# Autodesk Inventor assembly: DD
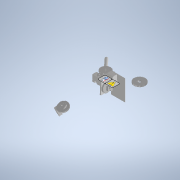
[picture p0: Inventor's stored thumbnail of the model, 180x180]
Saved by Autodesk Inventor 2020.2 (Build 242310000, 310)
## iProperties
Created: 2022-10-31
Part Number: DD
Document SubType Name: Assembly
Designer: Administrator
Author: Administrator
## Documents named in this file (14)
- C:\Users\Administrator\Documents\kamuy2\DD.iam
- C:\Users\Administrator\Documents\kamuy2\Parts\Part1.ipt
- C:\Users\Administrator\Documents\kamuy2\Parts\x-540_idle.ipt
- C:\Users\Administrator\Documents\kamuy2\Parts\XW540.N105.I101.ipt
- C:\Users\Administrator\Documents\kamuy2\Parts\GEABP1.0-80-10-A-20-KFC30-K3_Autodesk_Inventor_2020_20221101\AIS2020\GEABP1_0-80-10-A-20-KFC30-K3.iam
- C:\Users\Administrator\Documents\kamuy2\Parts\GEABP1.0-32-10-A-12-KFC22-K3_Autodesk_Inventor_2020_20221101\AIS2020\GEABP1_0-32-10-A-12-KFC22-K3.iam
- C:\Users\Administrator\Documents\kamuy2\Parts\Part2.ipt
- C:\Users\Administrator\Documents\kamuy2\Parts\Part5.ipt
- C:\Users\Administrator\Documents\kamuy2\Parts\BGHK6800VV-20_Autodesk_Inventor_2020_20221102\AIS2020\BGHK6800VV-20.iam
- C:\Users\Administrator\Documents\kamuy2\Parts\GEABP1.0-70-10-B-10-KFC30-K3_Autodesk_Inventor_2020_20221102\AIS2020\GEABP1_0-70-10-B-10-KFC30-K3.iam
- C:\Users\Administrator\Documents\kamuy2\Parts\Part7.ipt
- C:\Users\Administrator\Documents\kamuy2\Parts\C-SHA10_Autodesk_Inventor_2020_20221104\AIS2020\C-SHA10.iam
- C:\Users\Administrator\Documents\kamuy2\Parts\BGBFS6900DD-25_Autodesk_Inventor_2020_20221104\AIS2020\BGBFS6900DD-25.iam
- C:\Users\Administrator\Documents\kamuy2\Parts\Part8.ipt
## Components (20 placed, 13 different names)
1. Part1:1 — フラッシュ:1, メイト:1, フラッシュ:14, メイト:13, フラッシュ:15
2. x-540_idle:1 — メイト:4, メイト:5, メイト:33, フラッシュ:25, フラッシュ:26, メイト:47, フラッシュ:32
3. XW540.N105.I101:1 — フラッシュ:1, メイト:1, メイト:2, メイト:3, フラッシュ:14, メイト:19
4. GEABP1_0-32-10-A-12-KFC22-K3:1 [sub-assembly] — メイト:2, メイト:3, フラッシュ:22
5. GEABP1_0-32-10-A-12-KFC22-K3:2 [sub-assembly] — メイト:4, メイト:5, フラッシュ:23
6. Part2:1
7. x-540_idle:2
8. GEABP1_0-32-10-A-12-KFC22-K3:3 [sub-assembly] — フラッシュ:24
9. GEABP1_0-80-10-A-20-KFC30-K3:4 [sub-assembly]
10. Part5:1 — メイト:25, メイト:26, メイト:27, メイト:33, フラッシュ:25, フラッシュ:26, メイト:43, フラッシュ:32
11. BGHK6800VV-20:1 [sub-assembly] — メイト:13, フラッシュ:15, メイト:19, メイト:24
12. GEABP1_0-70-10-B-10-KFC30-K3:1 [sub-assembly] — フラッシュ:22, メイト:24, メイト:25, メイト:26, メイト:27
13. GEABP1_0-70-10-B-10-KFC30-K3:2 [sub-assembly] — フラッシュ:23, メイト:37, メイト:48, フラッシュ:34
14. GEABP1_0-70-10-B-10-KFC30-K3:3 [sub-assembly] — フラッシュ:24
15. Part7:1 — メイト:37, メイト:39, メイト:44, メイト:45, フラッシュ:34
16. C-SHA10:1 [sub-assembly] — フラッシュ:30, メイト:39, メイト:40, メイト:41, フラッシュ:33, メイト:49
17. C-SHA10:2 [sub-assembly] — フラッシュ:30, メイト:40, メイト:41
18. BGBFS6900DD-25:1 [sub-assembly] — メイト:43, メイト:44, フラッシュ:31, メイト:47
19. BGBFS6900DD-25:2 [sub-assembly] — フラッシュ:31, メイト:45, メイト:48, メイト:49
20. Part8:1 — フラッシュ:33
## Relationships (37: Mate 24, Flush 13)
- フラッシュ:1 [Flush]: Part1:1 ↔ XW540.N105.I101:1
- メイト:1 [Mate]: Part1:1 ↔ XW540.N105.I101:1
- メイト:2 [Mate]: XW540.N105.I101:1 ↔ GEABP1_0-32-10-A-12-KFC22-K3:1
- メイト:3 [Mate]: XW540.N105.I101:1 ↔ GEABP1_0-32-10-A-12-KFC22-K3:1
- メイト:4 [Mate]: x-540_idle:1 ↔ GEABP1_0-32-10-A-12-KFC22-K3:2
- メイト:5 [Mate]: x-540_idle:1 ↔ GEABP1_0-32-10-A-12-KFC22-K3:2
- [Mate]: x-540_idle:2 ↔ GEABP1_0-32-10-A-12-KFC22-K3:3
- [Mate]: x-540_idle:2 ↔ GEABP1_0-32-10-A-12-KFC22-K3:3
- フラッシュ:14 [Flush]: Part1:1 ↔ XW540.N105.I101:1
- メイト:13 [Mate]: Part1:1 ↔ BGHK6800VV-20:1
- フラッシュ:15 [Flush]: Part1:1 ↔ BGHK6800VV-20:1
- メイト:19 [Mate] (24 mm): XW540.N105.I101:1 ↔ BGHK6800VV-20:1
- フラッシュ:22 [Flush]: GEABP1_0-32-10-A-12-KFC22-K3:1 ↔ GEABP1_0-70-10-B-10-KFC30-K3:1
- メイト:24 [Mate]: BGHK6800VV-20:1 ↔ GEABP1_0-70-10-B-10-KFC30-K3:1
- メイト:25 [Mate]: Part5:1 ↔ GEABP1_0-70-10-B-10-KFC30-K3:1
- メイト:26 [Mate]: Part5:1 ↔ GEABP1_0-70-10-B-10-KFC30-K3:1
- メイト:27 [Mate]: Part5:1 ↔ GEABP1_0-70-10-B-10-KFC30-K3:1
- フラッシュ:23 [Flush]: GEABP1_0-32-10-A-12-KFC22-K3:2 ↔ GEABP1_0-70-10-B-10-KFC30-K3:2
- フラッシュ:24 [Flush]: GEABP1_0-32-10-A-12-KFC22-K3:3 ↔ GEABP1_0-70-10-B-10-KFC30-K3:3
- メイト:33 [Mate]: x-540_idle:1 ↔ Part5:1
- フラッシュ:25 [Flush]: x-540_idle:1 ↔ Part5:1
- フラッシュ:26 [Flush]: x-540_idle:1 ↔ Part5:1
- メイト:37 [Mate]: GEABP1_0-70-10-B-10-KFC30-K3:2 ↔ Part7:1
- フラッシュ:30 [Flush]: C-SHA10:1 ↔ C-SHA10:2
- メイト:39 [Mate]: Part7:1 ↔ C-SHA10:1
- メイト:40 [Mate]: C-SHA10:1 ↔ C-SHA10:2
- メイト:41 [Mate] (25 mm): C-SHA10:1 ↔ C-SHA10:2
- メイト:43 [Mate]: Part5:1 ↔ BGBFS6900DD-25:1
- メイト:44 [Mate]: Part7:1 ↔ BGBFS6900DD-25:1
- フラッシュ:31 [Flush]: BGBFS6900DD-25:1 ↔ BGBFS6900DD-25:2
- メイト:45 [Mate]: Part7:1 ↔ BGBFS6900DD-25:2
- メイト:47 [Mate] (17 mm): x-540_idle:1 ↔ BGBFS6900DD-25:1
- フラッシュ:32 [Flush]: x-540_idle:1 ↔ Part5:1
- フラッシュ:33 [Flush]: C-SHA10:1 ↔ Part8:1
- メイト:48 [Mate] (2 mm): GEABP1_0-70-10-B-10-KFC30-K3:2 ↔ BGBFS6900DD-25:2
- フラッシュ:34 [Flush]: GEABP1_0-70-10-B-10-KFC30-K3:2 ↔ Part7:1
- メイト:49 [Mate] (2 mm): C-SHA10:1 ↔ BGBFS6900DD-25:2
## Named parameters: d10_d5 = 0 mm, d11_d6 = 0 mm
